# Autodesk Inventor assembly: Recessed Wheels V1.0
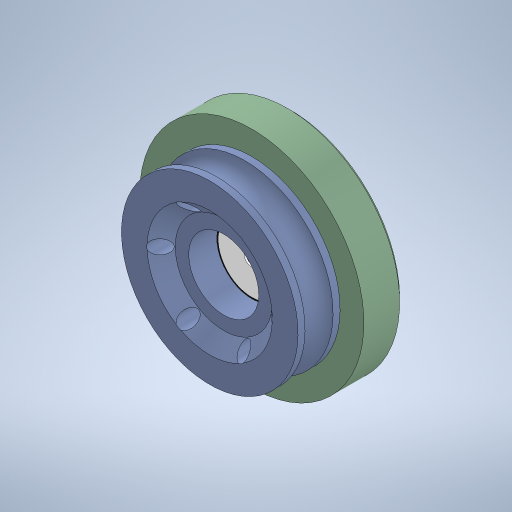
[picture p0: Inventor's stored thumbnail of the model, 512x512]
Saved by Autodesk Inventor 2023.2 (Build 272271000, 271)
## iProperties
Created: 2023-02-06
Part Number: Recessed Wheels V1.0
Document SubType Name: Assembly
Designer: Nathan Cai
Mass: 29.776 g
Surface Area: 113.605 cm^2
Volume: 23.0692 cm^3
Author: Nathan Cai
## Documents named in this file (6)
- E:\Documents\Inventor\Chort V2.0\Custom Wheel V2.0\Recessed Wheels V2.0.iam
- E:\Documents\Inventor\Chort V2.0\Custom Wheel V2.0\Tire Hub.ipt
- E:\Documents\Inventor\Chort V2.0\Custom Wheel V2.0\Tire.ipt
- E:\Documents\Inventor\Chort V2.0\Custom Wheel V2.0\T40_Hub_With_Retainer\T40_Hub_With_Retainer.iam
- E:\Documents\Inventor\Chort V2.0\Pulley.ipt
- E:\Documents\Inventor\Content Center Files\R2023\en-US\ANSI B18.6.3(27)\ANSI B18.6.3 - 6-32 UNC - 0.5(11).ipt
## Components (10 placed, 5 different names)
1. Tire Hub:1 — Flush:5, Mate:5, Mate:6, Mate:7, Flush:6, Mate:9, Mate:10, Mate:11, Mate:12, Mate:13, Mate:14, Mate:15, Mate:16, Mate:17, Mate:18, Mate:19, Mate:20, Mate:21, Mate:22
2. Tire:1 — Flush:5, Mate:5, Mate:8
3. T40_Hub_With_Retainer:1 [sub-assembly] — Mate:6, Mate:7, Flush:6
4. Pulley:1 — Mate:8, Mate:9, Mate:10
5. Cross Recessed Truss Head Machine Screw - Type I - Inch No. 6 - 32 - 1/2:1 — Mate:11, Mate:12
6. Cross Recessed Truss Head Machine Screw - Type I - Inch No. 6 - 32 - 1/2:2 — Mate:13, Mate:14
7. Cross Recessed Truss Head Machine Screw - Type I - Inch No. 6 - 32 - 1/2:3 — Mate:15, Mate:16
8. Cross Recessed Truss Head Machine Screw - Type I - Inch No. 6 - 32 - 1/2:4 — Mate:17, Mate:18
9. Cross Recessed Truss Head Machine Screw - Type I - Inch No. 6 - 32 - 1/2:5 — Mate:19, Mate:20
10. Cross Recessed Truss Head Machine Screw - Type I - Inch No. 6 - 32 - 1/2:6 — Mate:21, Mate:22
## Relationships (20: Mate 18, Flush 2)
- Flush:5: Tire Hub:1 ↔ Tire:1
- Mate:5: Tire Hub:1 ↔ Tire:1
- Mate:6: Tire Hub:1 ↔ T40_Hub_With_Retainer:1
- Mate:7 (0.0635 mm): Tire Hub:1 ↔ T40_Hub_With_Retainer:1
- Flush:6: Tire Hub:1 ↔ T40_Hub_With_Retainer:1
- Mate:8: Tire:1 ↔ Pulley:1
- Mate:9: Tire Hub:1 ↔ Pulley:1
- Mate:10: Tire Hub:1 ↔ Pulley:1
- Mate:11: Tire Hub:1 ↔ Cross Recessed Truss Head Machine Screw - Type I - Inch No. 6 - 32 - 1/2:1
- Mate:12: Tire Hub:1 ↔ Cross Recessed Truss Head Machine Screw - Type I - Inch No. 6 - 32 - 1/2:1
- Mate:13: Tire Hub:1 ↔ Cross Recessed Truss Head Machine Screw - Type I - Inch No. 6 - 32 - 1/2:2
- Mate:14: Tire Hub:1 ↔ Cross Recessed Truss Head Machine Screw - Type I - Inch No. 6 - 32 - 1/2:2
- Mate:15: Tire Hub:1 ↔ Cross Recessed Truss Head Machine Screw - Type I - Inch No. 6 - 32 - 1/2:3
- Mate:16: Tire Hub:1 ↔ Cross Recessed Truss Head Machine Screw - Type I - Inch No. 6 - 32 - 1/2:3
- Mate:17: Tire Hub:1 ↔ Cross Recessed Truss Head Machine Screw - Type I - Inch No. 6 - 32 - 1/2:4
- Mate:18: Tire Hub:1 ↔ Cross Recessed Truss Head Machine Screw - Type I - Inch No. 6 - 32 - 1/2:4
- Mate:19: Tire Hub:1 ↔ Cross Recessed Truss Head Machine Screw - Type I - Inch No. 6 - 32 - 1/2:5
- Mate:20: Tire Hub:1 ↔ Cross Recessed Truss Head Machine Screw - Type I - Inch No. 6 - 32 - 1/2:5
- Mate:21: Tire Hub:1 ↔ Cross Recessed Truss Head Machine Screw - Type I - Inch No. 6 - 32 - 1/2:6
- Mate:22: Tire Hub:1 ↔ Cross Recessed Truss Head Machine Screw - Type I - Inch No. 6 - 32 - 1/2:6
